# Autodesk Inventor assembly: mezzanineBoard
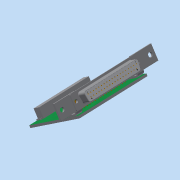
[picture p0: Inventor's stored thumbnail of the model, 180x180]
Saved by Autodesk Inventor 2016 (Build 200138000, 138)
## iProperties
Created: 2016-08-31
Part Number: mezzanineBoard
Document SubType Name: Assembly
Designer: Zara
Author: Zara
## Documents named in this file (6)
- C:\Users\Zara\Documents\hera-cad\Node\SNAP V2 enclosure release - pack-n-go export\SNAP V2 enclosure release - pack-n-go export\Workspaces\Workspace\components\mezzanineBoard.iam
- C:\Users\Zara\Documents\hera-cad\Node\SNAP V2 enclosure release - pack-n-go export\SNAP V2 enclosure release - pack-n-go export\Workspaces\Workspace\components\mezzaninePCB.ipt
- C:\Users\Zara\Documents\hera-cad\Node\SNAP V2 enclosure release - pack-n-go export\SNAP V2 enclosure release - pack-n-go export\Workspaces\Workspace\components\snapPinout.ipt
- C:\Users\Zara\Documents\hera-cad\Node\SNAP V2 enclosure release - pack-n-go export\SNAP V2 enclosure release - pack-n-go export\Workspaces\Workspace\components\174E-037-213.ipt
- C:\Users\Zara\Documents\hera-cad\Node\SNAP V2 enclosure release - pack-n-go export\SNAP V2 enclosure release - pack-n-go export\Workspaces\Workspace\components\dsub37Bracket_left.ipt
- C:\Users\Zara\Documents\hera-cad\Node\SNAP V2 enclosure release - pack-n-go export\SNAP V2 enclosure release - pack-n-go export\Workspaces\Workspace\components\dsub37Bracket_right.ipt
## Components (5 placed, 5 different names)
1. mezzaninePCB:1 — Mate:2, Flush:3, Flush:4, Mate:3, Mate:4
2. snapPinout:1 — Mate:2, Flush:3, Flush:4
3. 174E-037-213:1 — Mate:7, Mate:8, Mate:9, Mate:10
4. dsub37Bracket_left:1 — Mate:3, Mate:7, Mate:9
5. dsub37Bracket_right:1 — Mate:4, Mate:8, Mate:10
## Relationships (9: Mate 7, Flush 2)
- Mate:2: mezzaninePCB:1 ↔ snapPinout:1
- Flush:3: mezzaninePCB:1 ↔ snapPinout:1
- Flush:4 (9.3 mm): mezzaninePCB:1 ↔ snapPinout:1
- Mate:3: mezzaninePCB:1 ↔ dsub37Bracket_left:1
- Mate:4: mezzaninePCB:1 ↔ dsub37Bracket_right:1
- Mate:7: 174E-037-213:1 ↔ dsub37Bracket_left:1
- Mate:8: 174E-037-213:1 ↔ dsub37Bracket_right:1
- Mate:9: 174E-037-213:1 ↔ dsub37Bracket_left:1
- Mate:10: 174E-037-213:1 ↔ dsub37Bracket_right:1
